# Autodesk Inventor assembly: Gaveta
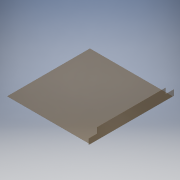
[picture p0: Inventor's stored thumbnail of the model, 180x180]
Saved by Autodesk Inventor 2018 (Build 220112000, 112)
## iProperties
Created: 2018-07-08
Part Number: Gaveta
Material: Genérico
Document SubType Name: Assembly
Designer: Regner
Author: Regner
## Documents named in this file (3)
- C:\Users\Regner\Documents\ROBOTA\2018\Tortura Ratos\Gaveta.iam
- C:\Users\Regner\Documents\ROBOTA\2018\Tortura Ratos\Tampa Gaveta.ipt
- C:\Users\Regner\Documents\ROBOTA\2018\Tortura Ratos\Fundo Gaveta.ipt
## Components (2 placed, 2 different names)
1. Tampa Gaveta:1 — Coincidência:1, Alinhamento:1, Alinhamento:2
2. Fundo Gaveta:1 — Coincidência:1, Alinhamento:1, Alinhamento:2
## Relationships (3: Flush 2, Mate 1)
- Coincidência:1 [Mate]: Tampa Gaveta:1 ↔ Fundo Gaveta:1
- Alinhamento:1 [Flush]: Tampa Gaveta:1 ↔ Fundo Gaveta:1
- Alinhamento:2 [Flush] (4.4 mm): Tampa Gaveta:1 ↔ Fundo Gaveta:1
